# Autodesk Inventor assembly: Tread Sproket Gear Assembly 2
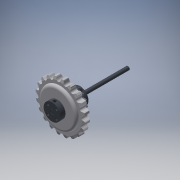
[picture p0: Inventor's stored thumbnail of the model, 180x180]
Saved by Autodesk Inventor 2016 (Build 200138000, 138)
## iProperties
Created: 2015-12-14
Part Number: Tread Sproket Gear Assembly 2
Document SubType Name: Assembly
Designer: tbloo
Author: tbloo
## Documents named in this file (6)
- C:\Users\TimB\Documents\GitHub\phi_robotics\3d-models\FTC_Tetrix_KOP_Block_Party\Tim Bloot Designs\JAr JaR Bot\Tread Sproket Gear Assembly 2.iam
- C:\Users\TimB\Documents\GitHub\phi_robotics\3d-models\FTC_Tetrix_KOP_Block_Party\Tetrix_Kit_FTC\Autodesk Inventor Files\tetrix_axle.ipt
- C:\Users\TimB\Documents\GitHub\phi_robotics\3d-models\FTC_Tetrix_KOP_Block_Party\Tetrix_Kit_FTC\Autodesk Inventor Files\tetrix_bushing.ipt
- C:\Users\TimB\Documents\GitHub\phi_robotics\3d-models\FTC_Tetrix_KOP_Block_Party\Tetrix_Kit_FTC\Autodesk Inventor Files\tetrix_tread_sprocket_2012.ipt
- C:\Users\TimB\Documents\GitHub\phi_robotics\3d-models\FTC_Tetrix_KOP_Block_Party\Tetrix_Kit_FTC\Autodesk Inventor Files\tetrix_axle_lock.iam
- C:\Users\TimB\Documents\GitHub\phi_robotics\3d-models\FTC_Tetrix_KOP_Block_Party\Tetrix_Kit_FTC\Autodesk Inventor Files\tetrix_chain_gear-16t.ipt
## Components (6 placed, 5 different names)
1. tetrix_axle:1 — Rigid:2
2. tetrix_tread_sprocket_2012:1 — Rotational:1, Rigid:1
3. tetrix_bushing:2 — Rotational:1, Rigid:4
4. tetrix_axle_lock:1 [sub-assembly] — Rigid:5
5. tetrix_axle_lock:2 [sub-assembly] — Rigid:1, Rigid:2
6. tetrix_chain_gear-16t:1 — Rigid:5, Rigid:4
## Relationships (5: WeldJoint 4, RevoluteJoint 1)
- Rotational:1 [RevoluteJoint]: tetrix_tread_sprocket_2012:1 ↔ tetrix_bushing:2
- Rigid:1 [WeldJoint]: tetrix_tread_sprocket_2012:1 ↔ tetrix_axle_lock:2
- Rigid:2 [WeldJoint]: tetrix_axle:1 ↔ tetrix_axle_lock:2
- Rigid:4 [WeldJoint]: tetrix_bushing:2 ↔ tetrix_chain_gear-16t:1
- Rigid:5 [WeldJoint]: tetrix_axle_lock:1 ↔ tetrix_chain_gear-16t:1
